# Autodesk Inventor assembly: plytka_nucleo_zlozenie
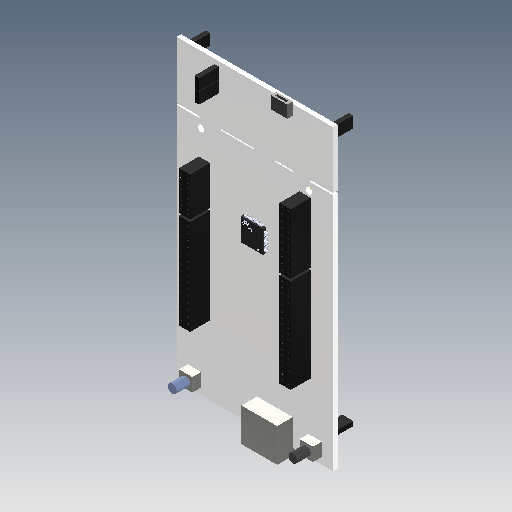
[picture p0: Inventor's stored thumbnail of the model, 512x512]
Saved by Autodesk Inventor 2021 (Build 250183000, 183)
## iProperties
Created: 2022-10-19
Part Number: plytka_nucleo_zlozenie
Document SubType Name: Assembly
Designer: agnpi
Author: agnpi
## Documents named in this file (3)
- D:\users\agnpi\Desktop\lekcje\SEMESTR VII\Inventor video\Zlozenie inne kolory\plytka_nucleo_zlozenie.iam
- D:\users\agnpi\Desktop\lekcje\SEMESTR VII\Inventor video\Zlozenie inne kolory\nucleo_746zg_.ipt
- D:\users\agnpi\Desktop\lekcje\SEMESTR VII\Inventor video\Zlozenie inne kolory\mikro.ipt
## Components (2 placed, 2 different names)
1. nucleo_746zg_:1 — Mate:1, Mate:2, Mate:3
2. mikro:1 — Mate:1, Mate:2, Mate:3
## Relationships (3: Mate 3)
- Mate:1: nucleo_746zg_:1 ↔ mikro:1
- Mate:2 (15 mm): nucleo_746zg_:1 ↔ mikro:1
- Mate:3 (-5 mm): nucleo_746zg_:1 ↔ mikro:1
